# Autodesk Inventor assembly: Assembly1
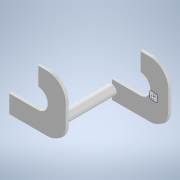
[picture p0: Inventor's stored thumbnail of the model, 180x180]
Saved by Autodesk Inventor 2020 (Build 240168000, 168)
## iProperties
Created: 2020-01-24
Part Number: Assembly1
Document SubType Name: Assembly
Designer: 1sfkeith
Author: 1sfkeith
## Documents named in this file (3)
- J:\Writable\Iron Riders\2020 Robot Parts\Assembly1.iam
- J:\Writable\Iron Riders\2020 Robot Parts\hook rod.ipt
- J:\Writable\Iron Riders\2020 Robot Parts\hook.ipt
## Components (3 placed, 2 different names)
1. hook rod:1 — Mate:1, Mate:2
2. hook:1 — Mate:1
3. hook:2 — Mate:2
## Relationships (2: Mate 2)
- Mate:1: hook rod:1 ↔ hook:1
- Mate:2: hook rod:1 ↔ hook:2
